# Autodesk Inventor assembly: 2x20
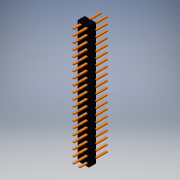
[picture p0: Inventor's stored thumbnail of the model, 180x180]
Saved by Autodesk Inventor 2016 (Build 200138000, 138)
## iProperties
Created: 2014-07-19
Part Number: 2x20
Document SubType Name: Assembly
Designer: Sawaiz Syed
Author: Sawaiz Syed
## Documents named in this file (3)
- C:\Users\Jonathan\Documents\Projects\dynodePiShield\coincidenceCounter\cad\electronics\2.54 breakaway\2x20.iam
- C:\Users\Jonathan\Documents\Projects\dynodePiShield\coincidenceCounter\cad\electronics\2.54 breakaway\Holder.ipt
- C:\Users\Jonathan\Documents\Projects\dynodePiShield\coincidenceCounter\cad\electronics\2.54 breakaway\Pin.ipt
## Components (80 placed, 2 different names)
1. Pin:1 — Mate:1, Mate:2, Flush:1
2. Holder:1 — Mate:1, Mate:2, Flush:1
3. Pin:2
4. Holder:2
5. Pin:3
6. Holder:3
7. Pin:4
8. Holder:4
9. Pin:5
10. Holder:5
11. Pin:6
12. Holder:6
13. Pin:7
14. Holder:7
15. Pin:8
16. Holder:8
17. Pin:9
18. Holder:9
19. Pin:10
20. Holder:10
21. Pin:11
22. Holder:11
23. Pin:12
24. Holder:12
25. Pin:13
26. Holder:13
27. Pin:14
28. Holder:14
29. Pin:15
30. Holder:15
31. Pin:16
32. Holder:16
33. Pin:17
34. Holder:17
35. Pin:18
36. Holder:18
37. Pin:19
38. Holder:19
39. Pin:20
40. Holder:20
41. Pin:21
42. Holder:21
43. Pin:22
44. Holder:22
45. Pin:23
46. Holder:23
47. Pin:24
48. Holder:24
49. Pin:25
50. Holder:25
51. Pin:26
52. Holder:26
53. Pin:27
54. Holder:27
55. Pin:28
56. Holder:28
57. Pin:29
58. Holder:29
59. Pin:30
60. Holder:30
61. Pin:31
62. Holder:31
63. Pin:32
64. Holder:32
65. Pin:33
66. Holder:33
67. Pin:34
68. Holder:34
69. Pin:35
70. Holder:35
71. Pin:36
72. Holder:36
73. Pin:37
74. Holder:37
75. Pin:38
76. Holder:38
77. Pin:39
78. Holder:39
79. Pin:40
80. Holder:40
## Component patterns: (40 elements, first: Pin:1 + Holder:1)
## Relationships (3: Mate 2, Flush 1)
- Mate:1: Pin:1 ↔ Holder:1
- Mate:2: Pin:1 ↔ Holder:1
- Flush:1 (-5.84 mm): Pin:1 ↔ Holder:1
